# Autodesk Inventor assembly: Rotor_Shaft_assembly
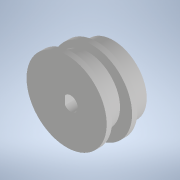
[picture p0: Inventor's stored thumbnail of the model, 180x180]
Saved by Autodesk Inventor 2021 (Build 250183000, 183)
## iProperties
Created: 2022-08-14
Part Number: Rotor_Shaft_assembly
Document SubType Name: Assembly
Designer: MicnedSQ
Author: MicnedSQ
## Documents named in this file (3)
- C:\Users\MicnedSQ\Desktop\V1\Rotor_Shaft_assembly.iam
- C:\Users\MicnedSQ\Desktop\V1\Rotor_shaft_2.ipt
- C:\Users\MicnedSQ\Desktop\V1\Rotor_shaft_2_2.ipt
## Components (2 placed, 2 different names)
1. Rotor_shaft_2:1 — Sztywne:1
2. Rotor_shaft_2_2:1 — Sztywne:1
## Relationships (1: WeldJoint 1)
- Sztywne:1 [WeldJoint]: Rotor_shaft_2:1 ↔ Rotor_shaft_2_2:1
